# Autodesk Inventor assembly: Assembly2
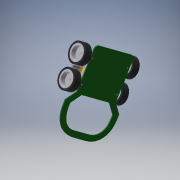
[picture p0: Inventor's stored thumbnail of the model, 180x180]
Saved by Autodesk Inventor 2016 (Build 200138000, 138)
## iProperties
Created: 2017-05-26
Part Number: Assembly2
Material: Ogólny
Document SubType Name: Assembly
Designer: Karol
Author: Karol
## Documents named in this file (14)
- D:\ele\MicroMouse\v2\Assembly2.iam
- D:\ele\MicroMouse\v2\wheel.ipt
- D:\ele\MicroMouse\v2\togh.ipt
- D:\ele\MicroMouse\v2\bolt.ipt
- D:\ele\MicroMouse\v2\tyre.ipt
- D:\ele\MicroMouse\v2\motor.ipt
- D:\ele\MicroMouse\v2\magnet.ipt
- D:\ele\MicroMouse\v2\mainpcb.ipt
- D:\ele\MicroMouse\v2\bolt_MIR1.ipt
- D:\ele\MicroMouse\v2\wheel_MIR1.ipt
- D:\ele\MicroMouse\v2\magnet_MIR1.ipt
- D:\ele\MicroMouse\v2\togh_MIR4.ipt
- D:\ele\MicroMouse\v2\tyre_MIR1.ipt
- D:\ele\MicroMouse\v2\motor_MIR3.ipt
## Components (19 placed, 13 different names)
1. mainpcb:1 — Rigid:37, Rigid:38
2. bolt:3 — Rotational:1
3. bolt:4 — Rotational:19
4. wheel:3
5. wheel:4
6. magnet:4
7. togh:2 — Rotational:19, Rigid:22, Rotational:1, Rigid:38
8. tyre:3
9. tyre:4
10. motor:2 — Rigid:22
11. bolt_MIR1:1 — Rigid:30, Rotational:23
12. bolt_MIR1:2 — Rigid:31, Rigid:33, Rotational:22
13. wheel_MIR1:1 — Rigid:30, Rigid:34
14. wheel_MIR1:2 — Rigid:31, Rigid:35
15. magnet_MIR1:2 — Rigid:33
16. togh_MIR4:1 — Rotational:22, Rotational:23, Rigid:36, Rigid:37
17. tyre_MIR1:1 — Rigid:34
18. tyre_MIR1:2 — Rigid:35
19. motor_MIR3:1 — Rigid:36
## Relationships (18: WeldJoint 14, RevoluteJoint 4)
- [WeldJoint]: bolt:4 ↔ wheel:4
- [WeldJoint]: bolt:3 ↔ wheel:3
- [WeldJoint]: bolt:4 ↔ magnet:4
- Rotational:19 [RevoluteJoint]: bolt:4 ↔ togh:2
- [WeldJoint]: wheel:3 ↔ tyre:3
- [WeldJoint]: wheel:4 ↔ tyre:4
- Rigid:22 [WeldJoint] (-0.5 mm): togh:2 ↔ motor:2
- Rotational:1 [RevoluteJoint]: bolt:3 ↔ togh:2
- Rigid:30 [WeldJoint]: bolt_MIR1:1 ↔ wheel_MIR1:1
- Rigid:31 [WeldJoint]: bolt_MIR1:2 ↔ wheel_MIR1:2
- Rigid:33 [WeldJoint]: bolt_MIR1:2 ↔ magnet_MIR1:2
- Rotational:22 [RevoluteJoint]: bolt_MIR1:2 ↔ togh_MIR4:1
- Rotational:23 [RevoluteJoint]: bolt_MIR1:1 ↔ togh_MIR4:1
- Rigid:34 [WeldJoint]: wheel_MIR1:1 ↔ tyre_MIR1:1
- Rigid:35 [WeldJoint]: wheel_MIR1:2 ↔ tyre_MIR1:2
- Rigid:36 [WeldJoint] (-0.5 mm): togh_MIR4:1 ↔ motor_MIR3:1
- Rigid:37 [WeldJoint]: mainpcb:1 ↔ togh_MIR4:1
- Rigid:38 [WeldJoint]: mainpcb:1 ↔ togh:2
## Named parameters: d102_d99 = 0 mm, d104_d101 = -0.5 mm, d105_d68 = 0 mm, d106_d67 = 0 mm, d107_d21 = -4.793458 deg, d108_d22 = -0.02503 mm, d111_d4 = 0 mm, d112_d5 = 0.127925 deg, d113_d6 = 0 mm, d114_d7 = -6.839272 deg, d117_d14 = 0 mm, d118_d15 = 2.56641 deg
